# Autodesk Inventor assembly: sharpener-concept-oneill
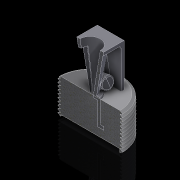
[picture p0: Inventor's stored thumbnail of the model, 180x180]
Saved by Autodesk Inventor 2019.3 (Build 233278000, 278)
## iProperties
Created: 2020-10-20
Part Number: sharpener-concept-oneill
Document SubType Name: Assembly
Designer: msokoliuk
Author: msokoliuk
## Documents named in this file (3)
- C:\SPEC19\sharpener-concept-oneill.iam
- C:\SPEC19\sharpener-concept-oneill.ipt
- C:\SPEC19\External-Components\Staedtler Sharpener.ipt
## Components (2 placed, 2 different names)
1. sharpener-concept-oneill:1 — Flush:1, Flush:2, Flush:3, Mate:5, Mate:6, Flush:8
2. Staedtler Sharpener:1 — Mate:5, Mate:6, Flush:8
## Relationships (6: Flush 4, Mate 2)
- Flush:1: sharpener-concept-oneill:1
- Flush:2: sharpener-concept-oneill:1
- Flush:3: sharpener-concept-oneill:1
- Mate:5: sharpener-concept-oneill:1 ↔ Staedtler Sharpener:1
- Mate:6: sharpener-concept-oneill:1 ↔ Staedtler Sharpener:1
- Flush:8 (-0.508 mm): sharpener-concept-oneill:1 ↔ Staedtler Sharpener:1
## Named parameters: SHR_EXP = 0.508 mm
